# Autodesk Inventor assembly: BoxBeam and Igus Mount
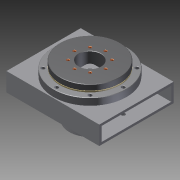
[picture p0: Inventor's stored thumbnail of the model, 180x180]
Saved by Autodesk Inventor 2015 (Build 190159000, 159)
## iProperties
Created: 2015-02-14
Part Number: BoxBeam and Igus Mount
Document SubType Name: Assembly
Designer: chapale16
Author: chapale16
## Documents named in this file (4)
- \\lhssvr02\Homedirs\Robotics Club\CAD Model 2015\Alternate Arm mounts\BoxBeam and Igus Mount.iam
- \\lhssvr02\Homedirs\Robotics Club\CAD Model 2015\Alternate Arm mounts\4x1x5 box beam.ipt
- \\lhssvr02\Homedirs\Robotics Club\CAD Model 2015\Game Components\The Tote Collector-Arms\Imported Components\PRT_01_30_1\PRT_01_30_1_MIR5.iam
- \\lhssvr02\Homedirs\Robotics Club\CAD Model 2015\Torque Limiter\TorqueLimiter.iam
## Components (3 placed, 3 different names)
1. 4x1x5 box beam:1 — Mate:2, Mate:3, Mate:4
2. PRT_01_30_1_MIR5:1 [sub-assembly] — Mate:2, Mate:3, Mate:4, Mate:5, Mate:6
3. TorqueLimiter:1 [sub-assembly] — Mate:5, Mate:6
## Relationships (5: Mate 5)
- Mate:2 (-50.8 mm): 4x1x5 box beam:1 ↔ PRT_01_30_1_MIR5:1
- Mate:3 (-63.5 mm): 4x1x5 box beam:1 ↔ PRT_01_30_1_MIR5:1
- Mate:4: 4x1x5 box beam:1 ↔ PRT_01_30_1_MIR5:1
- Mate:5: PRT_01_30_1_MIR5:1 ↔ TorqueLimiter:1
- Mate:6: PRT_01_30_1_MIR5:1 ↔ TorqueLimiter:1
